# Autodesk Inventor assembly: Plstic Box Rear A Assembly
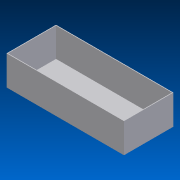
[picture p0: Inventor's stored thumbnail of the model, 180x180]
Saved by Autodesk Inventor 2012 (Build 160160000, 160)
## iProperties
Created: 2012-07-02
Part Number: Plstic Box Rear A Assembly
Document SubType Name: Assembly
Designer: Hemant
Author: Hemant
## Documents named in this file (4)
- C:\Users\Hemant\Documents\Pastic Box - Rear A\Plstic Box Rear A Assembly.iam
- C:\Users\Hemant\Documents\Pastic Box - Rear A\base.ipt
- C:\Users\Hemant\Documents\Pastic Box - Rear A\front face.ipt
- C:\Users\Hemant\Documents\Pastic Box - Rear A\side face.ipt
## Components (5 placed, 3 different names)
1. base:1 — Mate:1, Mate:2, Mate:3, Mate:4, Mate:5, Mate:6, Mate:7, Mate:8, Mate:9
2. front face:1 — Mate:2, Mate:7, Mate:10, Mate:11
3. front face:2 — Mate:4, Mate:5, Mate:9, Mate:12
4. side face:1 — Mate:3, Mate:8, Mate:10, Mate:12
5. side face:2 — Mate:1, Mate:6, Mate:11
## Relationships (12: Mate 12)
- Mate:1: base:1 ↔ side face:2
- Mate:2: base:1 ↔ front face:1
- Mate:3: base:1 ↔ side face:1
- Mate:4: base:1 ↔ front face:2
- Mate:5: base:1 ↔ front face:2
- Mate:6: base:1 ↔ side face:2
- Mate:7: base:1 ↔ front face:1
- Mate:8: base:1 ↔ side face:1
- Mate:9: base:1 ↔ front face:2
- Mate:10: front face:1 ↔ side face:1
- Mate:11: front face:1 ↔ side face:2
- Mate:12: front face:2 ↔ side face:1
